# Autodesk Inventor assembly: Голень в сборе
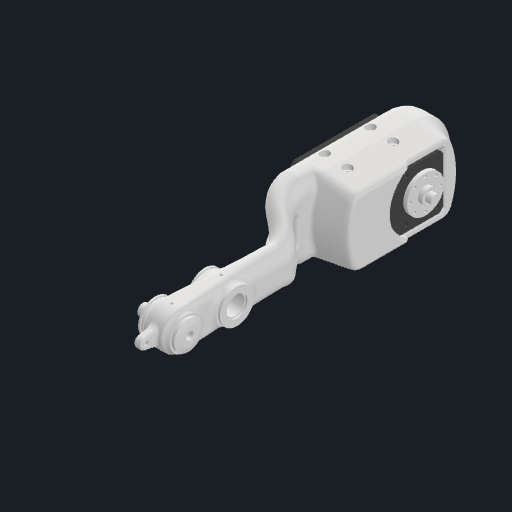
[picture p0: Inventor's stored thumbnail of the model, 512x512]
Saved by Autodesk Inventor 2025 (Build 290162010, 162A)
## iProperties
Created: 2024-12-05
Part Number: Голень в сборе
Document SubType Name: Assembly
Designer: Edward_Higgins
Author: Edward_Higgins
## Documents named in this file (5)
- D:\Users\Edward_Higgins\Desktop\ZAVOD\Робот Сколково\Голень в сборе.iam
- D:\Users\Edward_Higgins\Desktop\ZAVOD\Робот Сколково\DYNAMIXEL XM430-W350.ipt
- D:\Users\Edward_Higgins\Desktop\ZAVOD\Робот Сколково\Нога.ipt
- D:\Users\Edward_Higgins\Desktop\ZAVOD\Робот Сколково\Шайба.ipt
- D:\Users\Edward_Higgins\Desktop\ZAVOD\Робот Сколково\Ось односторонняя.ipt
## Components (6 placed, 4 different names)
1. DYNAMIXEL XM430-W350:1 — Совмещение:4, Совмещение:7, Совмещение:8
2. Нога:1 — Совмещение:6, Совмещение:7, Совмещение:8, Совмещение:20, Совмещение:21, Совмещение:26, Совмещение:30, Совмещение:31
3. Шайба:1 — Совмещение:21
4. Шайба:2 — Совмещение:20
5. Шайба:3 — Совмещение:29, Совмещение:31
6. Ось односторонняя:1 — Совмещение:26, Совмещение:29, Совмещение:30
## Relationships (10: Mate 10)
- Совмещение:4 [Mate]: DYNAMIXEL XM430-W350:1
- Совмещение:6 [Mate]: Нога:1
- Совмещение:7 [Mate] (0.25 mm): DYNAMIXEL XM430-W350:1 ↔ Нога:1
- Совмещение:8 [Mate]: DYNAMIXEL XM430-W350:1 ↔ Нога:1
- Совмещение:20 [Mate]: Нога:1 ↔ Шайба:2
- Совмещение:21 [Mate]: Нога:1 ↔ Шайба:1
- Совмещение:26 [Mate]: Нога:1 ↔ Ось односторонняя:1
- Совмещение:29 [Mate]: Шайба:3 ↔ Ось односторонняя:1
- Совмещение:30 [Mate]: Нога:1 ↔ Ось односторонняя:1
- Совмещение:31 [Mate]: Нога:1 ↔ Шайба:3
